# Autodesk Inventor assembly: Ensamble
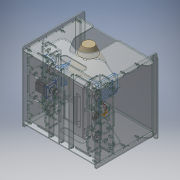
[picture p0: Inventor's stored thumbnail of the model, 180x180]
Saved by Autodesk Inventor 2019 (Build 230136000, 136)
## iProperties
Created: 2020-04-02
Part Number: Ensamble
Document SubType Name: Assembly
Designer: Jurgen
Author: Jurgen
## Documents named in this file (29)
- C:\Users\Jurgen\Documents\UN\PAI\Respirador_V1\Ensamble.iam
- C:\Users\Jurgen\Documents\UN\PAI\Respirador_V1\Base.ipt
- C:\Users\Jurgen\Documents\UN\PAI\Respirador_V1\Soporte_Motor.ipt
- C:\Users\Jurgen\Documents\UN\PAI\Respirador_V1\Soporte_Varilla_Lisa_Perpendicular\SHF8.ipt
- C:\Users\Jurgen\Documents\UN\PAI\Respirador_V1\Motor_Nema_17\BL17E19Motor.ipt
- C:\Users\Jurgen\Documents\UN\PAI\Respirador_V1\Soporte_Opuesto.ipt
- C:\Users\Jurgen\Documents\UN\Servomecanismos\Proyecto Academico\Modelo CAD V3.0\Rodamiento_ChumaceraKFL08.iam
- C:\Users\Jurgen\Documents\UN\PAI\Respirador_V1\Varilla_Lisa.ipt
- C:\Users\Jurgen\Documents\UN\PAI\Respirador_V1\Acoplamiento\Flexible Coupling 5mm x 8mm.ipt
- C:\Users\Jurgen\Documents\UN\PAI\Respirador_V1\Tornillo_Potencia.ipt
- C:\Users\Jurgen\Documents\UN\PAI\Respirador_V1\Corredera.ipt
- C:\Users\Jurgen\Documents\UN\Servomecanismos\Proyecto Academico\Modelo CAD V3.0\Tuerca_Tornillo de potencia.ipt
- C:\Users\Jurgen\Documents\UN\Servomecanismos\Proyecto Academico\Modelo CAD V3.0\LMF8UU.ipt
- C:\Users\Jurgen\Documents\UN\PAI\Respirador_V1\Ambu.ipt
- C:\Users\Jurgen\Documents\UN\PAI\Respirador_V1\Cubierta_Ducto_Motor.ipt
- C:\Users\Jurgen\Documents\UN\PAI\Respirador_V1\Mordaza.ipt
- C:\Users\Jurgen\Documents\UN\PAI\Respirador_V1\Cubierta_Rodamientos.ipt
- C:\Users\Jurgen\Documents\UN\PAI\Respirador_V1\Soporte_Ambu_Izq.ipt
- C:\Users\Jurgen\Documents\UN\PAI\Respirador_V1\Soporte_Ambu_Der.ipt
- C:\Users\Jurgen\Documents\UN\PAI\Respirador_V1\Soporte_Final_Carrera.ipt
- C:\Users\Jurgen\Documents\UN\PAI\Respirador_V1\Final_Carrera\Assembly - V-156-1C25 micro switch (Pressed).iam
- C:\Users\Jurgen\Documents\UN\PAI\Respirador_V1\Refuerzo_Conducto.ipt
- C:\Users\Jurgen\Documents\UN\PAI\Respirador_V1\Soporte_Ducto_Rod.ipt
- C:\Users\Jurgen\Documents\UN\PAI\Respirador_V1\Lat_Izq_Caja.ipt
- C:\Users\Jurgen\Documents\UN\PAI\Respirador_V1\Lat_Der_Caja.ipt
- C:\Users\Jurgen\Documents\UN\PAI\Respirador_V1\Tapa_Frontal.ipt
- C:\Users\Jurgen\Documents\UN\PAI\Respirador_V1\Tapa_Trasera.ipt
- C:\Users\Jurgen\Documents\UN\PAI\Respirador_V1\Tapa.ipt
- C:\Users\Jurgen\Documents\UN\PAI\Respirador_V1\Refuerzo_Base.ipt
## Components (38 placed, 28 different names)
1. BL17E19Motor:1 — Mate:7, Mate:8, Mate:9, Mate:27, Mate:57
2. SHF8:1 — Mate:10, Mate:11, Mate:12, Mate:26, Flush:2
3. SHF8:2 — Mate:13, Mate:14, Mate:15, Flush:1
4. SHF8:3 — Mate:16, Mate:17, Mate:18
5. SHF8:4 — Mate:19, Mate:20, Mate:21
6. Soporte_Motor:1 — Mate:7, Mate:8, Mate:9, Mate:10, Mate:11, Mate:12, Mate:13, Mate:14, Mate:15, Flush:3, Mate:41, Mate:42, Mate:62, Mate:63, Mate:79, Mate:81, Flush:19, Mate:83
7. Soporte_Opuesto:1 — Mate:16, Mate:17, Mate:18, Mate:19, Mate:20, Mate:21, Mate:25, Mate:28, Mate:54, Mate:55, Mate:56, Mate:58, Flush:5, Mate:59, Flush:14, Mate:68, Flush:15
8. Rodamiento_ChumaceraKFL08:1 [sub-assembly] — Mate:54, Mate:55, Mate:56
9. Varilla_Lisa:1 — Mate:25, Flush:1, Mate:52
10. Varilla_Lisa:2 — Mate:26, Flush:2, Mate:53
11. Flexible Coupling 5mm x 8mm:1 — Mate:27, Flush:3
12. Tornillo_Potencia:1 — Mate:28, Mate:57
13. Ambu:1 — Flush:13, Mate:66, Mate:67
14. Cubierta_Ducto_Motor:1 — Mate:41, Mate:42, Mate:60, Flush:10, Flush:12, Flush:16, Mate:69, Mate:70, Flush:17, Mate:71, Mate:79
15. Corredera:1 — Mate:43, Mate:44, Mate:45, Mate:46, Mate:47, Mate:48, Mate:49, Mate:50, Mate:51, Mate:53, Flush:9, Mate:64, Flush:11
16. LMF8UU:1 — Mate:46, Mate:47, Mate:48
17. LMF8UU:2 — Mate:49, Mate:50, Mate:51, Mate:52
18. Tuerca_Tornillo de potencia:1 — Mate:43, Mate:44, Mate:45
19. Base:1 — Mate:58, Flush:5, Mate:59, Mate:62, Mate:63, Flush:13, Flush:18, Mate:82, Flush:20, Mate:84, Flush:21, Mate:85, Mate:86, Flush:22, Mate:87, Flush:23, Mate:88, Mate:89, Flush:24, Mate:90, Mate:91, Mate:100, Mate:101, Mate:102
20. Mordaza:1 — Mate:60, Flush:10, Flush:12, Mate:66, Mate:67
21. Mordaza:2 — Flush:9, Mate:64, Flush:11
22. Cubierta_Rodamientos:1 — Flush:14, Mate:68, Flush:15, Mate:76, Mate:77, Mate:78, Mate:80
23. Soporte_Ambu_Izq:1 — Flush:16, Mate:69, Mate:70
24. Soporte_Ambu_Der:1 — Flush:17, Mate:71, Mate:80
25. Soporte_Final_Carrera:1 — Mate:73, Mate:74, Mate:75, Mate:76, Mate:77, Mate:78
26. Assembly - V-156-1C25 micro switch (Pressed):1 [sub-assembly] — Mate:73, Mate:74, Mate:75
27. Refuerzo_Conducto:2 — Mate:81, Flush:18, Mate:82
28. Refuerzo_Conducto:3 — Flush:19, Flush:20, Mate:83
29. Soporte_Ducto_Rod:1 — Mate:86, Flush:22, Mate:87
30. Soporte_Ducto_Rod:2 — Mate:84, Flush:21, Mate:85
31. Lat_Izq_Caja:1 — Flush:23, Mate:88, Mate:89, Mate:92, Mate:93, Mate:94, Flush:25, Mate:95, Mate:96, Flush:26, Flush:27, Flush:28, Flush:29, Flush:30, Flush:31
32. Lat_Der_Caja:1 — Flush:24, Mate:90, Mate:91
33. Tapa_Frontal:1 — Mate:92, Mate:93, Mate:94, Mate:97, Mate:98, Mate:99
34. Tapa_Trasera:1 — Flush:25, Mate:95, Mate:96
35. Tapa:1 — Mate:97, Mate:98, Mate:99
36. Refuerzo_Base:1 — Mate:101, Flush:28, Flush:31
37. Refuerzo_Base:2 — Mate:102, Flush:29, Flush:30
38. Refuerzo_Base:3 — Mate:100, Flush:26, Flush:27
## Relationships (105: Mate 78, Flush 27)
- Mate:7: BL17E19Motor:1 ↔ Soporte_Motor:1
- Mate:8: BL17E19Motor:1 ↔ Soporte_Motor:1
- Mate:9: BL17E19Motor:1 ↔ Soporte_Motor:1
- Mate:10: SHF8:1 ↔ Soporte_Motor:1
- Mate:11: SHF8:1 ↔ Soporte_Motor:1
- Mate:12: SHF8:1 ↔ Soporte_Motor:1
- Mate:13: SHF8:2 ↔ Soporte_Motor:1
- Mate:14: SHF8:2 ↔ Soporte_Motor:1
- Mate:15: SHF8:2 ↔ Soporte_Motor:1
- Mate:16: SHF8:3 ↔ Soporte_Opuesto:1
- Mate:17: SHF8:3 ↔ Soporte_Opuesto:1
- Mate:18: SHF8:3 ↔ Soporte_Opuesto:1
- Mate:19: SHF8:4 ↔ Soporte_Opuesto:1
- Mate:20: SHF8:4 ↔ Soporte_Opuesto:1
- Mate:21: SHF8:4 ↔ Soporte_Opuesto:1
- Mate:25: Soporte_Opuesto:1 ↔ Varilla_Lisa:1
- Flush:1: SHF8:2 ↔ Varilla_Lisa:1
- Mate:26: SHF8:1 ↔ Varilla_Lisa:2
- Flush:2: SHF8:1 ↔ Varilla_Lisa:2
- Mate:27: BL17E19Motor:1 ↔ Flexible Coupling 5mm x 8mm:1
- Flush:3 (-12 mm): Soporte_Motor:1 ↔ Flexible Coupling 5mm x 8mm:1
- Mate:28: Soporte_Opuesto:1 ↔ Tornillo_Potencia:1
- Mate:41: Soporte_Motor:1 ↔ Cubierta_Ducto_Motor:1
- Mate:42: Soporte_Motor:1 ↔ Cubierta_Ducto_Motor:1
- Mate:43: Corredera:1 ↔ Tuerca_Tornillo de potencia:1
- Mate:44: Corredera:1 ↔ Tuerca_Tornillo de potencia:1
- Mate:45: Corredera:1 ↔ Tuerca_Tornillo de potencia:1
- Mate:46: Corredera:1 ↔ LMF8UU:1
- Mate:47: Corredera:1 ↔ LMF8UU:1
- Mate:48: Corredera:1 ↔ LMF8UU:1
- Mate:49: Corredera:1 ↔ LMF8UU:2
- Mate:50: Corredera:1 ↔ LMF8UU:2
- Mate:51: Corredera:1 ↔ LMF8UU:2
- Mate:52: Varilla_Lisa:1 ↔ LMF8UU:2
- Mate:53: Varilla_Lisa:2 ↔ Corredera:1
- Mate:54: Soporte_Opuesto:1 ↔ Rodamiento_ChumaceraKFL08:1
- Mate:55: Soporte_Opuesto:1 ↔ Rodamiento_ChumaceraKFL08:1
- Mate:56: Soporte_Opuesto:1 ↔ Rodamiento_ChumaceraKFL08:1
- Mate:57 (1 mm): BL17E19Motor:1 ↔ Tornillo_Potencia:1
- Mate:58: Soporte_Opuesto:1 ↔ Base:1
- Flush:5: Soporte_Opuesto:1 ↔ Base:1
- Mate:59: Soporte_Opuesto:1 ↔ Base:1
- Mate:60: Cubierta_Ducto_Motor:1 ↔ Mordaza:1
- Flush:9: Corredera:1 ↔ Mordaza:2
- Flush:10: Cubierta_Ducto_Motor:1 ↔ Mordaza:1
- Mate:62: Soporte_Motor:1 ↔ Base:1
- Mate:63: Soporte_Motor:1 ↔ Base:1
- Mate:64: Corredera:1 ↔ Mordaza:2
- Flush:11: Corredera:1 ↔ Mordaza:2
- Flush:12 (55 mm): Cubierta_Ducto_Motor:1 ↔ Mordaza:1
- Flush:13: Ambu:1 ↔ Base:1
- Mate:66 (63.5 mm): Ambu:1 ↔ Mordaza:1
- Mate:67 (-50 mm): Ambu:1 ↔ Mordaza:1
- Flush:14: Soporte_Opuesto:1 ↔ Cubierta_Rodamientos:1
- Mate:68: Soporte_Opuesto:1 ↔ Cubierta_Rodamientos:1
- Flush:15: Soporte_Opuesto:1 ↔ Cubierta_Rodamientos:1
- Flush:16: Cubierta_Ducto_Motor:1 ↔ Soporte_Ambu_Izq:1
- Mate:69: Cubierta_Ducto_Motor:1 ↔ Soporte_Ambu_Izq:1
- Mate:70: Cubierta_Ducto_Motor:1 ↔ Soporte_Ambu_Izq:1
- Flush:17: Cubierta_Ducto_Motor:1 ↔ Soporte_Ambu_Der:1
- Mate:71: Cubierta_Ducto_Motor:1 ↔ Soporte_Ambu_Der:1
- Mate:73: Soporte_Final_Carrera:1 ↔ Assembly - V-156-1C25 micro switch (Pressed):1
- Mate:74: Soporte_Final_Carrera:1 ↔ Assembly - V-156-1C25 micro switch (Pressed):1
- Mate:75: Soporte_Final_Carrera:1 ↔ Assembly - V-156-1C25 micro switch (Pressed):1
- Mate:76: Cubierta_Rodamientos:1 ↔ Soporte_Final_Carrera:1
- Mate:77: Cubierta_Rodamientos:1 ↔ Soporte_Final_Carrera:1
- Mate:78: Cubierta_Rodamientos:1 ↔ Soporte_Final_Carrera:1
- Mate:79: Soporte_Motor:1 ↔ Cubierta_Ducto_Motor:1
- Mate:80: Cubierta_Rodamientos:1 ↔ Soporte_Ambu_Der:1
- Mate:81: Soporte_Motor:1 ↔ Refuerzo_Conducto:2
- Flush:18: Base:1 ↔ Refuerzo_Conducto:2
- Mate:82: Base:1 ↔ Refuerzo_Conducto:2
- Flush:19: Soporte_Motor:1 ↔ Refuerzo_Conducto:3
- Flush:20: Base:1 ↔ Refuerzo_Conducto:3
- Mate:83: Soporte_Motor:1 ↔ Refuerzo_Conducto:3
- Mate:84: Base:1 ↔ Soporte_Ducto_Rod:2
- Flush:21: Base:1 ↔ Soporte_Ducto_Rod:2
- Mate:85: Base:1 ↔ Soporte_Ducto_Rod:2
- Mate:86: Base:1 ↔ Soporte_Ducto_Rod:1
- Flush:22: Base:1 ↔ Soporte_Ducto_Rod:1
- Mate:87: Base:1 ↔ Soporte_Ducto_Rod:1
- Flush:23: Base:1 ↔ Lat_Izq_Caja:1
- Mate:88: Base:1 ↔ Lat_Izq_Caja:1
- Mate:89: Base:1 ↔ Lat_Izq_Caja:1
- Flush:24: Base:1 ↔ Lat_Der_Caja:1
- Mate:90: Base:1 ↔ Lat_Der_Caja:1
- Mate:91: Base:1 ↔ Lat_Der_Caja:1
- Mate:92: Lat_Izq_Caja:1 ↔ Tapa_Frontal:1
- Mate:93: Lat_Izq_Caja:1 ↔ Tapa_Frontal:1
- Mate:94: Lat_Izq_Caja:1 ↔ Tapa_Frontal:1
- Flush:25: Lat_Izq_Caja:1 ↔ Tapa_Trasera:1
- Mate:95: Lat_Izq_Caja:1 ↔ Tapa_Trasera:1
- Mate:96: Lat_Izq_Caja:1 ↔ Tapa_Trasera:1
- Mate:97: Tapa_Frontal:1 ↔ Tapa:1
- Mate:98: Tapa_Frontal:1 ↔ Tapa:1
- Mate:99: Tapa_Frontal:1 ↔ Tapa:1
- Mate:100: Base:1 ↔ Refuerzo_Base:3
- Flush:26: Lat_Izq_Caja:1 ↔ Refuerzo_Base:3
- Flush:27: Lat_Izq_Caja:1 ↔ Refuerzo_Base:3
- Mate:101: Base:1 ↔ Refuerzo_Base:1
- Flush:28: Lat_Izq_Caja:1 ↔ Refuerzo_Base:1
- Mate:102: Base:1 ↔ Refuerzo_Base:2
- Flush:29: Lat_Izq_Caja:1 ↔ Refuerzo_Base:2
- Flush:30: Lat_Izq_Caja:1 ↔ Refuerzo_Base:2
- Flush:31: Lat_Izq_Caja:1 ↔ Refuerzo_Base:1
